# Autodesk Inventor assembly: chain tensioner
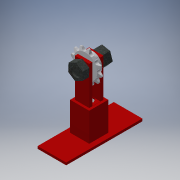
[picture p0: Inventor's stored thumbnail of the model, 180x180]
Saved by Autodesk Inventor 2016 (Build 200138000, 138)
## iProperties
Created: 2016-01-17
Part Number: chain tensioner
Document SubType Name: Assembly
Designer: gus
Mass: 118.105 g
Surface Area: 304.925 cm^2
Volume: 48.927 cm^3
Density: 2.4139 g/cm^3
Author: gus
## Documents named in this file (5)
- \\Mac\Home\Desktop\1510-stronghold-CAD-master\chassis\chain tensioner\chain tensioner.iam
- \\Mac\Home\Desktop\1510-stronghold-CAD-master\chassis\chain tensioner\mounting plate.ipt
- \\Mac\Home\Desktop\1510-stronghold-CAD-master\chassis\chain tensioner\slider.iam
- \\Mac\Home\Desktop\1510-stronghold-CAD-master\chassis\chain tensioner\10-32 bolt.ipt
- \\Mac\Home\Desktop\1510-stronghold-CAD-master\chassis\chain tensioner\10-32 nut.ipt
## Components (4 placed, 4 different names)
1. mounting plate:1 — Cylindrical:1, Mate:1, Mate:3
2. slider:1 [sub-assembly] — Cylindrical:2, Mate:1, Mate:2
3. 10-32 bolt:1 — Cylindrical:1, Cylindrical:2, Cylindrical:3, Mate:3
4. 10-32 nut:1 — Cylindrical:3, Mate:2
## Relationships (6: CylindricalJoint 3, Mate 3)
- Cylindrical:1: mounting plate:1 ↔ 10-32 bolt:1
- Cylindrical:2: slider:1 ↔ 10-32 bolt:1
- Cylindrical:3: 10-32 bolt:1 ↔ 10-32 nut:1
- Mate:1: mounting plate:1 ↔ slider:1
- Mate:2: slider:1 ↔ 10-32 nut:1
- Mate:3: mounting plate:1 ↔ 10-32 bolt:1
